# Autodesk Inventor assembly: full guns 2
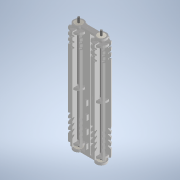
[picture p0: Inventor's stored thumbnail of the model, 180x180]
Saved by Autodesk Inventor 2020.1 (Build 241239000, 239)
## iProperties
Created: 2022-03-19
Part Number: full guns 2
Document SubType Name: Assembly
Designer: User
Author: User
## Documents named in this file (5)
- D:\GitHub\TANK\3D-turret\full guns 2.iam
- D:\GitHub\TANK\3D-turret\gun.iam
- D:\GitHub\TANK\3D-turret\соединение пушек.ipt
- D:\GitHub\TANK\3D-turret\подшипник.ipt
- D:\GitHub\TANK\3D-turret\центр пушки.ipt
## Components (9 placed, 4 different names)
1. gun:2 [sub-assembly] — С поворотом:1
2. gun:3 [sub-assembly] — С поворотом:2
3. соединение пушек:1 — Жесткий:1, Жесткий:2, Жесткий:3
4. подшипник:1 — Жесткий:1, С поворотом:2
5. подшипник:2 — Жесткий:2, С поворотом:1
6. центр пушки:1 — Жесткий:3, Жесткий:6
7. соединение пушек:2 — Жесткий:6
8. подшипник:3
9. подшипник:4
## Relationships (8: WeldJoint 6, RevoluteJoint 2)
- Жесткий:1 [WeldJoint]: соединение пушек:1 ↔ подшипник:1
- Жесткий:2 [WeldJoint]: соединение пушек:1 ↔ подшипник:2
- С поворотом:1 [RevoluteJoint]: gun:2 ↔ подшипник:2
- С поворотом:2 [RevoluteJoint]: gun:3 ↔ подшипник:1
- Жесткий:3 [WeldJoint]: соединение пушек:1 ↔ центр пушки:1
- [WeldJoint]: соединение пушек:2 ↔ подшипник:3
- [WeldJoint]: соединение пушек:2 ↔ подшипник:4
- Жесткий:6 [WeldJoint]: центр пушки:1 ↔ соединение пушек:2
## Named parameters: d10_d0 = 0 mm, d11_d1 = 0 mm
